# Autodesk Inventor assembly: Interfas_2
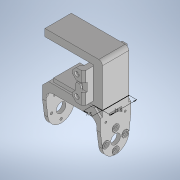
[picture p0: Inventor's stored thumbnail of the model, 180x180]
Saved by Autodesk Inventor 2021.3 (Build 253353000, 353)
## iProperties
Created: 2022-01-30
Part Number: Interfas_2
Document SubType Name: Assembly
Designer: epm01
Author: epm01
## Documents named in this file (3)
- D:\Archivos\2020-2\Papime\Banco_serial\Interfas_2.iam
- D:\Archivos\2020-2\Papime\Banco_serial\Bracket_bas.ipt
- D:\Archivos\2020-2\Papime\Banco_serial\FP04-F3.ipt
## Components (2 placed, 2 different names)
1. Bracket_bas:1 — Coincidencia:1, Coincidencia:2, Nivelación:1
2. FP04-F3:1 — Coincidencia:1, Coincidencia:2, Nivelación:1
## Relationships (3: Mate 2, Flush 1)
- Coincidencia:1 [Mate]: Bracket_bas:1 ↔ FP04-F3:1
- Coincidencia:2 [Mate]: Bracket_bas:1 ↔ FP04-F3:1
- Nivelación:1 [Flush] (-8.1 mm): Bracket_bas:1 ↔ FP04-F3:1
